# Autodesk Inventor assembly: 4212
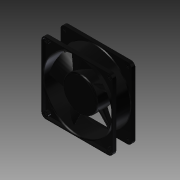
[picture p0: Inventor's stored thumbnail of the model, 180x180]
Saved by Autodesk Inventor 2014 (Build 180170000, 170)
## iProperties
Shininess: 64.0
Angle Display Precision: 2
Document Length Units: 11272
Document Angle Units: 11279
Document Time Units: 11290
Document Mass Units: 11286
Document Length Units Precision: 3
Document Angle Units Precision: 2
Category: Electrical
Company: Autodesk Inc.
Created: 2014-01-01
Part Number: 4212
Document SubType Name: Assembly
Designer: Autodesk Inc.
Catalog Web Link: http://www.ebmpapst.us/allpdfs/4200.PDF
Description: Compact fan (Large)
Vendor: ebmpabst
Density: 0.0
Volumn: 0.0
Area: 0.0
PropertySet Name: Model Information
Control State: 0
Master: False
Checked Out: False
Author: Autodesk Inc.
## Documents named in this file (3)
- D:\Data Folder\FIRST 2014\KOP Parts\Electrical\ELEC_FanLarge_4212.iam
- D:\Data Folder\FIRST 2014\KOP Parts\Electrical\Parts\Fan Housing.ipt
- D:\Data Folder\FIRST 2014\KOP Parts\Electrical\Parts\fan.ipt
## Components (2 placed, 2 different names)
1. Fan Housing:1 — Flush:1, Mate:1, Mate:2
2. fan:1 — Flush:1, Mate:1, Mate:2
## Relationships (3: Mate 2, Flush 1)
- Flush:1: Fan Housing:1 ↔ fan:1
- Mate:1: Fan Housing:1 ↔ fan:1
- Mate:2: Fan Housing:1 ↔ fan:1
